# Autodesk Inventor assembly: 足ユニット
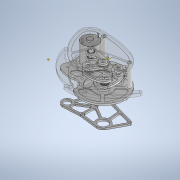
[picture p0: Inventor's stored thumbnail of the model, 180x180]
Saved by Autodesk Inventor 2022.2 (Build 262287010, 287A)
## iProperties
Created: 2022-01-10
Part Number: 足ユニット
Document SubType Name: Assembly
Designer: acps
Author: acps
## Documents named in this file (12)
- C:\Users\acps\Documents\srdc\srdc_ksh\脚\足ユニット.iam
- C:\Users\acps\Documents\srdc\srdc_ksh\脚\足(単独).iam
- C:\Users\acps\Documents\srdc\srdc_ksh\脚\足外フレーム.ipt
- C:\Users\acps\Documents\srdc\srdc_ksh\脚\足内フレーム.ipt
- C:\Users\acps\Documents\srdc\srdc_ksh\スペーサ\l40.ipt
- C:\Users\acps\Documents\srdc\srdc_ksh\カム\カム4.ipt
- C:\Users\acps\Documents\srdc\srdc_ksh\オイレス\w5f15-17n.ipt
- C:\Users\acps\Documents\srdc\srdc_ksh\モータ\M-RS-380.ipt
- C:\Users\acps\Documents\srdc\srdc_ksh\脚\ギア抑え.ipt
- C:\Users\acps\Documents\srdc\srdc_ksh\脚\モータマウント.ipt
- C:\Users\acps\Documents\srdc\srdc_ksh\ベアリング\Φ6-12a.ipt
- C:\Users\acps\Documents\srdc\srdc_ksh\スペーサ\l5.ipt
## Components (13 placed, 11 different names)
1. 足外フレーム:1 — Insert:2, Insert:7, Mate:21, Insert:14
2. 足(単独):1 [sub-assembly] — Mate:19, Mate:20, Mate:21, Mate:23, Mate:24, Mate:25, Insert:12, Mate:26, Insert:13, Insert:15
3. 足内フレーム:1 — Mate:4, Insert:8, Mate:10, Mate:14, Mate:15, Insert:10, Insert:11, Mate:22
4. l40:1 — Insert:2, Mate:22
5. l40:2 — Insert:7, Insert:8
6. l40:3 — Mate:19, Mate:20, Insert:11
7. カム4:1 — Mate:4, Insert:9, Mate:23, Mate:24, Mate:25, Insert:12
8. w5f15-17n:1 — Insert:9
9. M-RS-380:1 — Mate:10, Mate:16, Mate:17, Mate:18
10. ギア抑え:1
11. モータマウント:1 — Mate:14, Mate:15, Insert:10, Mate:16, Mate:17, Mate:18
12. Φ6-12a:1 — Mate:26, Insert:13, Insert:14
13. l5:1 — Insert:15
## Relationships (25: Mate 15, Insert 10)
- Insert:2: 足外フレーム:1 ↔ l40:1
- Mate:4: 足内フレーム:1 ↔ カム4:1
- Insert:7: 足外フレーム:1 ↔ l40:2
- Insert:8: 足内フレーム:1 ↔ l40:2
- Insert:9: カム4:1 ↔ w5f15-17n:1
- Mate:10: 足内フレーム:1 ↔ M-RS-380:1
- Mate:14: 足内フレーム:1 ↔ モータマウント:1
- Mate:15: 足内フレーム:1 ↔ モータマウント:1
- Insert:10: 足内フレーム:1 ↔ モータマウント:1
- Mate:16: M-RS-380:1 ↔ モータマウント:1
- Mate:17: M-RS-380:1 ↔ モータマウント:1
- Mate:18: M-RS-380:1 ↔ モータマウント:1
- Mate:19: 足(単独):1 ↔ l40:3
- Mate:20: 足(単独):1 ↔ l40:3
- Mate:21: 足外フレーム:1 ↔ 足(単独):1
- Insert:11: 足内フレーム:1 ↔ l40:3
- Mate:22: 足内フレーム:1 ↔ l40:1
- Mate:23: 足(単独):1 ↔ カム4:1
- Mate:24: 足(単独):1 ↔ カム4:1
- Mate:25: 足(単独):1 ↔ カム4:1
- Insert:12: 足(単独):1 ↔ カム4:1
- Mate:26: 足(単独):1 ↔ Φ6-12a:1
- Insert:13: 足(単独):1 ↔ Φ6-12a:1
- Insert:14: 足外フレーム:1 ↔ Φ6-12a:1
- Insert:15: 足(単独):1 ↔ l5:1
